# Autodesk Inventor assembly: upper long wall
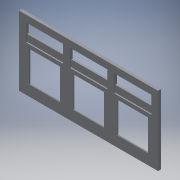
[picture p0: Inventor's stored thumbnail of the model, 180x180]
Saved by Autodesk Inventor 2017 (Build 210142000, 142)
## iProperties
Created: 2019-05-06
Part Number: upper long wall
Document SubType Name: Assembly
Designer: Roman
Author: Roman
## Documents named in this file (6)
- C:\Users\Roman\Documents\CAD\tegu rev2\upper walls\window wall\upper window wall.iam
- C:\Users\Roman\Documents\CAD\tegu rev2\upper walls\window wall\upper window wall h bar.ipt
- C:\Users\Roman\Documents\CAD\tegu rev2\upper walls\window wall\upper window wall v bar.ipt
- C:\Users\Roman\Documents\CAD\tegu rev2\upper walls\long wall\upper long wall back new.ipt
- C:\Users\Roman\Documents\CAD\tegu rev2\upper walls\window wall\window rev2\window frame.iam
- C:\Users\Roman\Documents\CAD\tegu rev2\upper walls\window wall\upper window wall h bar short.ipt
## Components (13 placed, 5 different names)
1. upper window wall h bar:1 — Mate:1, Flush:1, Flush:2, Mate:3, Flush:5, Flush:6, Flush:7, Mate:4, Mate:6, Mate:7
2. upper window wall h bar:2 — Mate:2, Flush:3, Flush:4
3. upper long wall back new:1 — Mate:3, Flush:5, Flush:6
4. window frame:1 [sub-assembly] — Flush:7, Mate:4, Mate:5, Mate:15
5. window frame:2 [sub-assembly] — Flush:8, Mate:6, Mate:8, Mate:14
6. window frame:3 [sub-assembly] — Flush:9, Mate:7, Mate:9, Mate:13
7. upper window wall h bar short:1 — Mate:10, Mate:15, Flush:10
8. upper window wall h bar short:2 — Mate:11, Mate:14, Flush:11
9. upper window wall h bar short:3 — Mate:12, Mate:13, Flush:12
10. upper window wall v bar:1 — Mate:1, Flush:1, Flush:2, Mate:2, Flush:3, Flush:4, Mate:5, Mate:10
11. upper window wall v bar:2 — Flush:8, Mate:11, Flush:10, Flush:11
12. upper window wall v bar:3 — Flush:9, Mate:8, Mate:12, Flush:12
13. upper window wall v bar:4 — Mate:9
## Component patterns: (4 elements, first: upper window wall v bar:1)
## Relationships (27: Mate 15, Flush 12)
- Mate:1: upper window wall h bar:1 ↔ upper window wall v bar:1
- Flush:1: upper window wall h bar:1 ↔ upper window wall v bar:1
- Flush:2: upper window wall h bar:1 ↔ upper window wall v bar:1
- Mate:2: upper window wall h bar:2 ↔ upper window wall v bar:1
- Flush:3: upper window wall h bar:2 ↔ upper window wall v bar:1
- Flush:4: upper window wall h bar:2 ↔ upper window wall v bar:1
- Mate:3: upper window wall h bar:1 ↔ upper long wall back new:1
- Flush:5: upper window wall h bar:1 ↔ upper long wall back new:1
- Flush:6: upper window wall h bar:1 ↔ upper long wall back new:1
- Flush:7: upper window wall h bar:1 ↔ window frame:1
- Mate:4: upper window wall h bar:1 ↔ window frame:1
- Mate:5: window frame:1 ↔ upper window wall v bar:1
- Flush:8: window frame:2 ↔ upper window wall v bar:2
- Flush:9: window frame:3 ↔ upper window wall v bar:3
- Mate:6: upper window wall h bar:1 ↔ window frame:2
- Mate:7: upper window wall h bar:1 ↔ window frame:3
- Mate:8: window frame:2 ↔ upper window wall v bar:3
- Mate:9: window frame:3 ↔ upper window wall v bar:4
- Mate:10: upper window wall h bar short:1 ↔ upper window wall v bar:1
- Mate:11: upper window wall h bar short:2 ↔ upper window wall v bar:2
- Mate:12: upper window wall h bar short:3 ↔ upper window wall v bar:3
- Mate:13: window frame:3 ↔ upper window wall h bar short:3
- Mate:14: window frame:2 ↔ upper window wall h bar short:2
- Mate:15: window frame:1 ↔ upper window wall h bar short:1
- Flush:10: upper window wall h bar short:1 ↔ upper window wall v bar:2
- Flush:11: upper window wall h bar short:2 ↔ upper window wall v bar:2
- Flush:12: upper window wall h bar short:3 ↔ upper window wall v bar:3
